# Autodesk Inventor assembly: PCBA_estimation_20190215
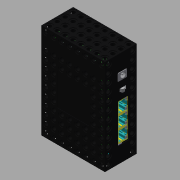
[picture p0: Inventor's stored thumbnail of the model, 180x180]
Saved by Autodesk Inventor 2019.3 (Build 233278000, 278)
## iProperties
Created: 2019-02-15
Part Number: PCBA_estimation_20190215
Document SubType Name: Assembly
Designer: Varga Daniel
Sending System: SolidWorks 2018
Last Author: david
Last Saved: 2019-02-15
Author: Varga Daniel
## Documents named in this file (12)
- C:\!_Dani\!_cloud\OneDrive\!_munka\Revolution\RevvyDemoKit\Structural parts\Demo parts\BrainSofteq\Inventor imported\PCBA_estimation_20190215.iam
- C:\!_Dani\!_cloud\OneDrive\!_munka\Revolution\RevvyDemoKit\Structural parts\Demo parts\BrainSofteq\Inventor imported\17x8669_2213145-2.ipt
- C:\!_Dani\!_cloud\OneDrive\!_munka\Revolution\RevvyDemoKit\Structural parts\Demo parts\BrainSofteq\Inventor imported\BRcA.ipt
- C:\!_Dani\!_cloud\OneDrive\!_munka\Revolution\RevvyDemoKit\Structural parts\Demo parts\BrainSofteq\Inventor imported\Micro SD Card.ipt
- C:\!_Dani\!_cloud\OneDrive\!_munka\Revolution\RevvyDemoKit\Structural parts\Demo parts\BrainSofteq\Inventor imported\JHY_813270_2000mAh.ipt
- C:\!_Dani\!_cloud\OneDrive\!_munka\Revolution\RevvyDemoKit\Structural parts\Demo parts\BrainSofteq\Inventor imported\Power_Jack_2mm.ipt
- C:\!_Dani\!_cloud\OneDrive\!_munka\Revolution\RevvyDemoKit\Structural parts\Demo parts\BrainSofteq\Inventor imported\PR(E,P)C020DAAN-RC.ipt
- C:\!_Dani\!_cloud\OneDrive\!_munka\Revolution\RevvyDemoKit\Structural parts\Demo parts\BrainSofteq\Inventor imported\SHR-05V-S-B.ipt
- C:\!_Dani\!_cloud\OneDrive\!_munka\Revolution\RevvyDemoKit\Structural parts\Demo parts\BrainSofteq\Inventor imported\RapberryPiZero_Shrinkwrap.ipt
- C:\!_Dani\!_cloud\OneDrive\!_munka\Revolution\RevvyDemoKit\Structural parts\Demo parts\BrainSofteq\Inventor imported\RRRC_carrier_board_Shrinkwrap.ipt
- C:\!_Dani\!_cloud\OneDrive\!_munka\Revolution\RevvyDemoKit\Structural parts\Demo parts\BrainSofteq\Inventor imported\RRRC_LED_board_Shrinkwrap.ipt
- C:\!_Dani\!_cloud\OneDrive\!_munka\Revolution\RevvyDemoKit\Structural parts\Demo parts\Microphone_hole_plug.ipt
## Components (20 placed, 11 different names)
1. RapberryPiZero_Shrinkwrap:1
2. RRRC_carrier_board_Shrinkwrap:1
3. RRRC_LED_board_Shrinkwrap:1
4. 17x8669_2213145-2:1
5. 17x8669_2213145-2:2
6. 17x8669_2213145-2:3
7. 17x8669_2213145-2:4
8. 17x8669_2213145-2:5
9. 17x8669_2213145-2:6
10. 17x8669_2213145-2:7
11. 17x8669_2213145-2:8
12. 17x8669_2213145-2:9
13. 17x8669_2213145-2:10
14. BRcA:1 — Flush:1, Flush:2
15. Micro SD Card:1
16. JHY_813270_2000mAh:1
17. Power_Jack_2mm:1
18. PR(E,P)C020DAAN-RC:1
19. SHR-05V-S-B:1
20. Microphone_hole_plug:1 — Flush:1, Flush:2
## Relationships (2: Flush 2)
- Flush:1: BRcA:1 ↔ Microphone_hole_plug:1
- Flush:2: BRcA:1 ↔ Microphone_hole_plug:1
